# Autodesk Inventor assembly: Module with Cover
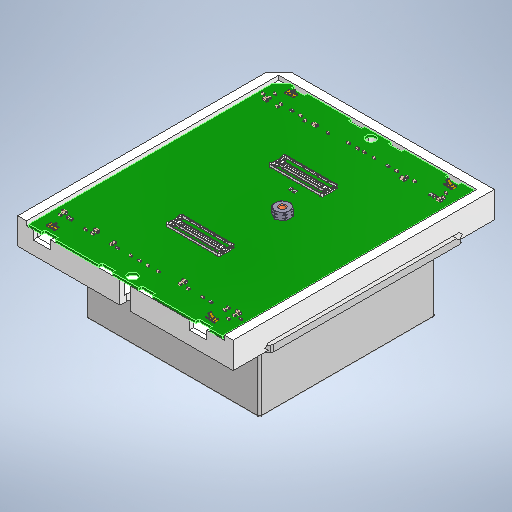
[picture p0: Inventor's stored thumbnail of the model, 512x512]
Saved by Autodesk Inventor 2025 (Build 290162000, 162)
## iProperties
Created: 2025-02-28
Part Number: Module with Cover
Document SubType Name: Assembly
Designer: Caleb Fangmeier
Author: Caleb Fangmeier
## Documents named in this file (5)
- C:\Users\cfang\Desktop\nebraska-silicon-lab\Hardware\ETL\Module Assembly\Digital Module Cover V3\Module with Cover.iam
- C:\Users\cfang\Desktop\nebraska-silicon-lab\Hardware\ETL\Module Assembly\Digital Module Cover V3\Digital Module Cover V3.ipt
- C:\Users\cfang\Desktop\nebraska-silicon-lab\Hardware\ETL\modules\tamale v1.5\Module PCB V1b\Module PCB V1b.ipt
- C:\Users\cfang\Desktop\nebraska-silicon-lab\Hardware\ETL\Module Assembly\Digital Module Cover V3\Installation Tool 1.ipt
- C:\Users\cfang\Desktop\nebraska-silicon-lab\Hardware\ETL\Module Assembly\Digital Module Cover V3\Installation Tool Collar.ipt
## Components (4 placed, 4 different names)
1. Digital Module Cover V3:1 — Mate:1, Mate:2, Mate:3, Mate:4, Mate:5
2. Module PCB V1b:1 — Mate:1, Mate:2
3. Installation Tool 1:1 — Mate:6, Mate:7
4. Installation Tool Collar:1 — Mate:3, Mate:4, Mate:5, Mate:6, Mate:7
## Relationships (7: Mate 7)
- Mate:1: Digital Module Cover V3:1 ↔ Module PCB V1b:1
- Mate:2: Digital Module Cover V3:1 ↔ Module PCB V1b:1
- Mate:3: Digital Module Cover V3:1 ↔ Installation Tool Collar:1
- Mate:4 (0.1 mm): Digital Module Cover V3:1 ↔ Installation Tool Collar:1
- Mate:5 (0.1 mm): Digital Module Cover V3:1 ↔ Installation Tool Collar:1
- Mate:6 (0.1 mm): Installation Tool 1:1 ↔ Installation Tool Collar:1
- Mate:7 (0.1 mm): Installation Tool 1:1 ↔ Installation Tool Collar:1
